# Autodesk Inventor assembly: Base stand BZB 550-900mm BVL3-H=550
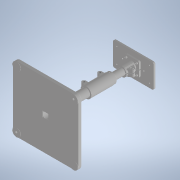
[picture p0: Inventor's stored thumbnail of the model, 180x180]
Saved by Autodesk Inventor 2021 (Build 250183000, 183)
## iProperties
Category: PARTsolutions
Company: RNA
Created: 2025-06-23
Part Number: Base stand BZB 550-900mm BVL3-H=550
Catalog Web Link: www.cadenas.de
Description: Base stand BZB-Accessories
Vendor: RNA
Document SubType Name: Assembly
Designer: psAdmin
Manufacturer: RNA
Mass: 5239.45 g
Surface Area: 8250.03 cm^2
Volume: 5239.45 cm^3
Density: 1 g/cm^3
Title: 31000133
Author: Cadenas PARTsolutions
Comments: Accessories
PSOL_IDENT_0: {$CADENAS_DATA/23d-libs/rna/bunker/zubehoer/bzb_asmtab.prj},208 {VTYP=3D},{STYP=ASSTAB},{NB=Base sta
PSOL_IDENT_1: nd BZB 550-900mm BVL3-H=550},{LINA=31000133},{NN=Base stand BZB},{DATE=14.03.2019 16:37:46},{GEOMDAT
PSOL_IDENT_2: E=14.03.2019 16:37:40},{VERSION=},{LINEID=200},{WBVAR=H},{WBNUMERIC=H}  {NB=Base stand BZB 550-900mm
PSOL_IDENT_3: BVL3-H=550},{LINA=31000133},{KT=DUMMY},{CNSORDERNO=31000133},{KOMP=Bodenstaender BZB 550-900mm BVL3
PSOL_IDENT_4: },{BTYP=BVL3},{HMIN=550},{HMAX=900},{H=550},{PPATH=assemblies/bzb_asmtpl.prj},{XTXT=Base stand BZB 5
PSOL_IDENT_5: 50-900mm BVL3},{ROW=1}
NB: Base stand BZB 550-900mm BVL3-H=550
NN: Base stand BZB
NT: Accessories
NBSYN: $XTXT.-H=$H.
LINA: 31000133
CATALOG: Rhein-Nadel-Automation
CNSORDERNO: 31000133
KOMP: Base stand BZB 550-900mm BVL3
BTYP: BVL3
H: 550
SUPPLIER: RNA
ARTICLENO: Base stand BZB 550-900mm BVL3-H=550
BOMINFO: 31000133
CREATOR: CADENAS GmbH
## Documents named in this file (8)
- e:\temp\worker_COMMON_405\temp\tmp_196_42_PaILy\format_0\Base stand BZB 550-900mm BVL3-H=550.iam
- e:\temp\worker_COMMON_405\temp\tmp_196_42_PaILy\format_0\BZB-FP.ipt
- e:\temp\worker_COMMON_405\temp\tmp_196_42_PaILy\format_0\BZB-PDOWN.ipt
- e:\temp\worker_COMMON_405\temp\tmp_196_42_PaILy\format_0\BZB-MFK.ipt
- e:\temp\worker_COMMON_405\temp\tmp_196_42_PaILy\format_0\31000133profil_up(550).ipt
- e:\temp\worker_COMMON_405\temp\tmp_196_42_PaILy\format_0\BZA-GP.ipt
- e:\temp\worker_COMMON_405\temp\tmp_196_42_PaILy\format_0\31000133platte.ipt
- e:\temp\worker_COMMON_405\temp\tmp_196_42_PaILy\format_0\M10x30.ipt
## Components (7 placed, 7 different names)
1. BZB-FP:1 — PROFIL_XY@1 <-> S1_DOWN_XY@2, PROFIL_Z@1 <-> S1_DOWN_Z@2, PROFIL_YZ@1 <-> S1_DOWN_YZ@2, PROFIL2_Z@1 <-> S2_DOWN_Z@4, PROFIL2_YZ@1 <-> S2_DOWN_YZ@4
2. BZB-PDOWN:1 — PROFIL_XY@1 <-> S1_DOWN_XY@2, PROFIL_Z@1 <-> S1_DOWN_Z@2, PROFIL_YZ@1 <-> S1_DOWN_YZ@2, S1_UP_XY@2 <-> KLEMM_XY@3, S1_UP_Z@2 <-> KLEMM_Z@3, S1_UP_YZ@2 <-> KLEMM_YZ@3
3. BZB-MFK:1 — S1_UP_XY@2 <-> KLEMM_XY@3, S1_UP_Z@2 <-> KLEMM_Z@3, S1_UP_YZ@2 <-> KLEMM_YZ@3
4. 31000133profil_up(550):1 — PROFIL2_Z@1 <-> S2_DOWN_Z@4, PROFIL2_YZ@1 <-> S2_DOWN_YZ@4, S2_UP_XY@4 <-> PROFIL_XY@5, S2_UP_Z@4 <-> PROFIL_Z@5, S2_UP_YZ@4 <-> PROFIL_YZ@5
5. BZA-GP:1 — S2_UP_XY@4 <-> PROFIL_XY@5, S2_UP_Z@4 <-> PROFIL_Z@5, S2_UP_YZ@4 <-> PROFIL_YZ@5, DUMMY_XY@5 <-> PLATTE_XY@6, DUMMY_Z@5 <-> PLATTE_Z@6, DUMMY_YZ@5 <-> PLATTE_YZ@6, SCHRAUBE_XY@5 <-> SCHRAUBE_XY@7, SCHRAUBE_Z@5 <-> SCHRAUBE_Z@7, SCHRAUBE_YZ@5 <-> SCHRAUBE_YZ@7
6. 31000133platte:1 — DUMMY_XY@5 <-> PLATTE_XY@6, DUMMY_Z@5 <-> PLATTE_Z@6, DUMMY_YZ@5 <-> PLATTE_YZ@6
7. M10x30:1 — SCHRAUBE_XY@5 <-> SCHRAUBE_XY@7, SCHRAUBE_Z@5 <-> SCHRAUBE_Z@7, SCHRAUBE_YZ@5 <-> SCHRAUBE_YZ@7
## Relationships (17: Mate 11, Angle 6)
- PROFIL_XY@1 <-> S1_DOWN_XY@2 [Mate]: BZB-FP:1 ↔ BZB-PDOWN:1
- PROFIL_Z@1 <-> S1_DOWN_Z@2 [Mate]: BZB-FP:1 ↔ BZB-PDOWN:1
- PROFIL_YZ@1 <-> S1_DOWN_YZ@2 [Angle] (0 deg): BZB-FP:1 ↔ BZB-PDOWN:1
- S1_UP_XY@2 <-> KLEMM_XY@3 [Mate]: BZB-PDOWN:1 ↔ BZB-MFK:1
- S1_UP_Z@2 <-> KLEMM_Z@3 [Mate]: BZB-PDOWN:1 ↔ BZB-MFK:1
- S1_UP_YZ@2 <-> KLEMM_YZ@3 [Angle] (0 deg): BZB-PDOWN:1 ↔ BZB-MFK:1
- PROFIL2_Z@1 <-> S2_DOWN_Z@4 [Mate]: BZB-FP:1 ↔ 31000133profil_up(550):1
- PROFIL2_YZ@1 <-> S2_DOWN_YZ@4 [Angle] (0 deg): BZB-FP:1 ↔ 31000133profil_up(550):1
- S2_UP_XY@4 <-> PROFIL_XY@5 [Mate]: 31000133profil_up(550):1 ↔ BZA-GP:1
- S2_UP_Z@4 <-> PROFIL_Z@5 [Mate]: 31000133profil_up(550):1 ↔ BZA-GP:1
- S2_UP_YZ@4 <-> PROFIL_YZ@5 [Angle] (180 deg): 31000133profil_up(550):1 ↔ BZA-GP:1
- DUMMY_XY@5 <-> PLATTE_XY@6 [Mate]: BZA-GP:1 ↔ 31000133platte:1
- DUMMY_Z@5 <-> PLATTE_Z@6 [Mate]: BZA-GP:1 ↔ 31000133platte:1
- DUMMY_YZ@5 <-> PLATTE_YZ@6 [Angle] (180 deg): BZA-GP:1 ↔ 31000133platte:1
- SCHRAUBE_XY@5 <-> SCHRAUBE_XY@7 [Mate]: BZA-GP:1 ↔ M10x30:1
- SCHRAUBE_Z@5 <-> SCHRAUBE_Z@7 [Mate]: BZA-GP:1 ↔ M10x30:1
- SCHRAUBE_YZ@5 <-> SCHRAUBE_YZ@7 [Angle] (0 deg): BZA-GP:1 ↔ M10x30:1
